# Autodesk Inventor assembly: Igus and Arm Bracket
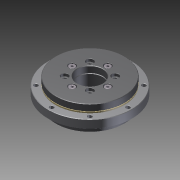
[picture p0: Inventor's stored thumbnail of the model, 180x180]
Saved by Autodesk Inventor 2015 (Build 190159000, 159)
## iProperties
Created: 2015-01-19
Part Number: Igus and Arm Bracket
Document SubType Name: Assembly
Designer: chapale16
Author: chapale16
## Documents named in this file (4)
- \\lhssvr02\Homedirs\Robotics Club\CAD Model 2015\Igus and Arm Bracket.iam
- \\lhssvr02\Homedirs\Robotics Club\CAD Model 2015\Game Components\The Tote Collector-Arms\Imported Components\PRT_01_30_1\PRT_01_30_1.iam
- \\lhssvr02\Homedirs\Robotics Club\CAD Model 2015\Game Components\The Tote Collector-Arms\P60 Gear Box_MIR2_MIR.ipt
- \\lhssvr02\Homedirs\Robotics Club\CAD Model 2015\Alternate Arm mounts\lbeam final_MIR.ipt
## Components (3 placed, 3 different names)
1. PRT_01_30_1:1 [sub-assembly] — Mate:1, Mate:2
2. P60 Gear Box_MIR2_MIR:1 — Mate:1, Mate:2, Mate:3, Mate:4
3. lbeam final_MIR:1 — Mate:3, Mate:4
## Relationships (4: Mate 4)
- Mate:1: PRT_01_30_1:1 ↔ P60 Gear Box_MIR2_MIR:1
- Mate:2: PRT_01_30_1:1 ↔ P60 Gear Box_MIR2_MIR:1
- Mate:3: P60 Gear Box_MIR2_MIR:1 ↔ lbeam final_MIR:1
- Mate:4: P60 Gear Box_MIR2_MIR:1 ↔ lbeam final_MIR:1
